# Autodesk Inventor assembly: ABD_RIGHT_OP
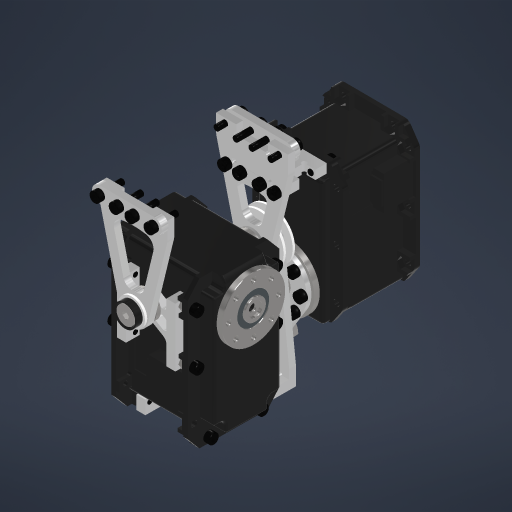
[picture p0: Inventor's stored thumbnail of the model, 512x512]
Saved by Autodesk Inventor 2024.3 (Build 283343000, 343)
## iProperties
Created: 2024-01-25
Part Number: ABD_RIGHT_OP
Document SubType Name: Assembly
Designer: ASUS
Mass: 367.451 g
Surface Area: 648.88 cm^2
Volume: 184.634 cm^3
Author: ASUS
## Documents named in this file (21)
- C:\Users\ASUS\Desktop\Anti_Backlash_Structure_OP\v1_Frame\ABD_RIGHT_OP.iam
- C:\Users\ASUS\Desktop\Anti_Backlash_Structure_OP\v1_Frame\Roll_Fixation_R.ipt
- C:\Users\ASUS\Desktop\Anti_Backlash_Structure_OP\v1_Frame\Slider_crank_horn.ipt
- C:\Users\ASUS\Desktop\Anti_Backlash_Structure_OP\v1_Frame\Roll_Fixation_L.ipt
- C:\Users\ASUS\Desktop\Anti_Backlash_Structure_OP\v1_Frame\Roll_Fixation_Frame.ipt
- C:\Users\ASUS\Desktop\Anti_Backlash_Structure_OP\v1_Frame\Leg_joint_slider_frame.ipt
- C:\Users\ASUS\Desktop\Anti_Backlash_Structure_OP\v1_Frame\Roll_Fixation_Frame_Back.ipt
- C:\Users\ASUS\Desktop\Anti_Backlash_Structure_OP\v1_Frame\106_Slider_Fixation.ipt
- C:\Users\ASUS\Desktop\Anti_Backlash_Structure_OP\v1_Frame\hip joint fix washer.ipt
- C:\Users\ASUS\Desktop\Anti_Backlash_Structure_OP\v1_Frame\Roll_Fixation_Frameto64.ipt
- C:\Users\ASUS\Desktop\ABD_2024_Eindhoven\MISUMI\Roll_Fixation_Frame_8mm_Set.iam
- C:\Users\ASUS\Desktop\ABD_2024_Eindhoven\MISUMI\CSH-ST-M2_5-8_203.ipt
- C:\Users\ASUS\Desktop\ABD_2024_Eindhoven\MISUMI\hip_joint_fix_washer_10mm_Set.iam
- C:\Users\ASUS\Desktop\Anti_Backlash_Structure_OP\MISUMI\ABD_4mm_set.iam
- C:\Users\ASUS\Desktop\Anti_Backlash_Structure_OP\v1_Frame\Front_Frame_Fixer.iam
- C:\Users\ASUS\Desktop\Anti_Backlash_Structure_OP\v1_Frame\Rear_Frame_Fixer.iam
- C:\Users\ASUS\Desktop\Anti_Backlash_Structure_OP\v1_Frame\Crank_Slider_Fixer.iam
- C:\Users\ASUS\Desktop\Anti_Backlash_Structure_OP\ROBOTIS(Inventor 2024 ver.)\DXL\MX-106T+idle.ipt.iam
- C:\Users\ASUS\Desktop\Anti_Backlash_Structure_OP\ROBOTIS(Inventor 2024 ver.)\DXL\MX-64T.ipt
- C:\Users\ASUS\Desktop\ABD_2024_Eindhoven\ROBOTIS(Inventor 2024 ver.)\HORN\64-106Horn.ipt
- MX-106T+idle.ipt
## Components (30 placed, 19 different names)
1. Roll_Fixation_R:1 — 메이트:51, 각도:1, 삽입:2, 삽입:24, 메이트:76
2. Slider_crank_horn:1 — 삽입:3, 삽입:20, 메이트:69, 삽입:29, 메이트:82
3. Roll_Fixation_L:1 — 메이트:52, 각도:2, 삽입:4, 메이트:77
4. Roll_Fixation_Frame:1 — 메이트:51, 메이트:54
5. Leg_joint_slider_frame:1 — 메이트:53, 삽입:17, 삽입:18, 메이트:63, 메이트:83
6. Roll_Fixation_Frame_Back:1 — 메이트:52, 메이트:53, 플러쉬:1, 삽입:13, 삽입:16, 각도:3, 삽입:23
7. 106_Slider_Fixation:1 — 메이트:72, 메이트:73, 메이트:74
8. hip joint fix washer:1 — 삽입:5, 메이트:55
9. hip joint fix washer:2 — 삽입:6, 메이트:56
10. Roll_Fixation_Frameto64:1 — 플러쉬:1, 삽입:14, 삽입:15, 메이트:66, 메이트:68, 메이트:80, 메이트:81
11. Roll_Fixation_Frame_8mm_Set:1 [sub-assembly] — 메이트:77, 메이트:78, 삽입:25
12. Roll_Fixation_Frame_8mm_Set:2 [sub-assembly] — 삽입:22, 메이트:75
13. CSH-ST-M2_5-8_203:1 — 삽입:18
14. CSH-ST-M2_5-8_203:2 — 삽입:17
15. Roll_Fixation_Frame_8mm_Set:3 [sub-assembly] — 삽입:26, 메이트:79
16. hip_joint_fix_washer_10mm_Set:1 [sub-assembly] — 삽입:5, 메이트:55
17. hip_joint_fix_washer_10mm_Set:2 [sub-assembly] — 삽입:6, 메이트:56
18. CSH-ST-M2_5-8_203:3 — 삽입:15
19. CSH-ST-M2_5-8_203:4 — 삽입:13
20. CSH-ST-M2_5-8_203:5 — 삽입:14
21. CSH-ST-M2_5-8_203:6 — 삽입:16
22. Front_Frame_Fixer:1 [sub-assembly] — 각도:1, 삽입:2, 메이트:54
23. Rear_Frame_Fixer:1 [sub-assembly] — 각도:2, 삽입:4, 삽입:23
24. Crank_Slider_Fixer:1 [sub-assembly] — 삽입:3, 메이트:63, 메이트:83
25. CSH-ST-M2_5-8_203:7 — 메이트:66, 삽입:27
26. CSH-ST-M2_5-8_203:8 — 메이트:68, 삽입:28
27. ABD_4mm_set:1 [sub-assembly] — 삽입:20, 메이트:69
28. MX-106T+idle.ipt:1 [sub-assembly] — 메이트:72, 메이트:73, 메이트:74, 삽입:22, 메이트:75, 삽입:24, 메이트:76, 메이트:78, 삽입:25, 삽입:26, 메이트:79
29. MX-64T:1 — 메이트:80, 메이트:81, 삽입:27, 삽입:28
30. 64-106Horn:1 — 삽입:29, 메이트:82
## Relationships (59: Mate 34, Insert 21, Angle 3, Flush 1)
- [Mate]: Roll_Fixation_Frame:1 ↔ Roll_Fixation_Frame_Back:1
- [Mate]: Leg_joint_slider_frame:1 ↔ 106_Slider_Fixation:1
- [Mate]: Leg_joint_slider_frame:1 ↔ 106_Slider_Fixation:1
- [Mate]: Leg_joint_slider_frame:1 ↔ 106_Slider_Fixation:1
- [Mate]: Roll_Fixation_Frame:1 ↔ hip joint fix washer:1
- [Mate]: Roll_Fixation_Frame:1 ↔ hip joint fix washer:1
- [Mate]: Roll_Fixation_Frame:1 ↔ hip joint fix washer:1
- [Mate]: Roll_Fixation_Frame_Back:1 ↔ hip joint fix washer:2
- [Mate]: Roll_Fixation_Frame_Back:1 ↔ hip joint fix washer:2
- [Mate]: Roll_Fixation_Frame_Back:1 ↔ hip joint fix washer:2
- [Mate]: Roll_Fixation_Frame_Back:1 ↔ Roll_Fixation_Frameto64:1
- [Mate]: Roll_Fixation_Frame_Back:1 ↔ Roll_Fixation_Frameto64:1
- 메이트:51 [Mate]: Roll_Fixation_R:1 ↔ Roll_Fixation_Frame:1
- 메이트:52 [Mate]: Roll_Fixation_L:1 ↔ Roll_Fixation_Frame_Back:1
- 메이트:53 [Mate]: Leg_joint_slider_frame:1 ↔ Roll_Fixation_Frame_Back:1
- 각도:1 [Angle] (0 deg): Roll_Fixation_R:1 ↔ Front_Frame_Fixer:1
- 삽입:2 [Insert]: Roll_Fixation_R:1 ↔ Front_Frame_Fixer:1
- 삽입:3 [Insert]: Slider_crank_horn:1 ↔ Crank_Slider_Fixer:1
- 각도:2 [Angle] (0 deg): Roll_Fixation_L:1 ↔ Rear_Frame_Fixer:1
- 삽입:4 [Insert]: Roll_Fixation_L:1 ↔ Rear_Frame_Fixer:1
- 메이트:54 [Mate]: Roll_Fixation_Frame:1 ↔ Front_Frame_Fixer:1
- 삽입:5 [Insert]: hip joint fix washer:1 ↔ hip_joint_fix_washer_10mm_Set:1
- 메이트:55 [Mate]: hip joint fix washer:1 ↔ hip_joint_fix_washer_10mm_Set:1
- 삽입:6 [Insert]: hip joint fix washer:2 ↔ hip_joint_fix_washer_10mm_Set:2
- 메이트:56 [Mate]: hip joint fix washer:2 ↔ hip_joint_fix_washer_10mm_Set:2
- 플러쉬:1 [Flush]: Roll_Fixation_Frame_Back:1 ↔ Roll_Fixation_Frameto64:1
- 삽입:13 [Insert]: Roll_Fixation_Frame_Back:1 ↔ CSH-ST-M2_5-8_203:4
- 삽입:14 [Insert]: Roll_Fixation_Frameto64:1 ↔ CSH-ST-M2_5-8_203:5
- 삽입:15 [Insert]: Roll_Fixation_Frameto64:1 ↔ CSH-ST-M2_5-8_203:3
- 삽입:16 [Insert]: Roll_Fixation_Frame_Back:1 ↔ CSH-ST-M2_5-8_203:6
- 삽입:17 [Insert]: Leg_joint_slider_frame:1 ↔ CSH-ST-M2_5-8_203:2
- 삽입:18 [Insert]: Leg_joint_slider_frame:1 ↔ CSH-ST-M2_5-8_203:1
- 메이트:63 [Mate]: Leg_joint_slider_frame:1 ↔ Crank_Slider_Fixer:1
- 메이트:66 [Mate]: Roll_Fixation_Frameto64:1 ↔ CSH-ST-M2_5-8_203:7
- 메이트:68 [Mate]: Roll_Fixation_Frameto64:1 ↔ CSH-ST-M2_5-8_203:8
- 삽입:20 [Insert]: Slider_crank_horn:1 ↔ ABD_4mm_set:1
- 메이트:69 [Mate]: Slider_crank_horn:1 ↔ ABD_4mm_set:1
- 각도:3 [Angle] (0 deg): Roll_Fixation_Frame_Back:1
- [Insert] (0.5 mm): MX-64T:1 ↔ 64-106Horn:1
- 메이트:72 [Mate]: 106_Slider_Fixation:1 ↔ MX-106T+idle.ipt:1
- 메이트:73 [Mate]: 106_Slider_Fixation:1 ↔ MX-106T+idle.ipt:1
- 메이트:74 [Mate] (0.5 mm): 106_Slider_Fixation:1 ↔ MX-106T+idle.ipt:1
- 삽입:22 [Insert]: Roll_Fixation_Frame_8mm_Set:2 ↔ MX-106T+idle.ipt:1
- 메이트:75 [Mate]: Roll_Fixation_Frame_8mm_Set:2 ↔ MX-106T+idle.ipt:1
- 삽입:23 [Insert]: Roll_Fixation_Frame_Back:1 ↔ Rear_Frame_Fixer:1
- 삽입:24 [Insert] (0.5 mm): Roll_Fixation_R:1 ↔ MX-106T+idle.ipt:1
- 메이트:76 [Mate]: Roll_Fixation_R:1 ↔ MX-106T+idle.ipt:1
- 메이트:77 [Mate]: Roll_Fixation_L:1 ↔ Roll_Fixation_Frame_8mm_Set:1
- 메이트:78 [Mate]: Roll_Fixation_Frame_8mm_Set:1 ↔ MX-106T+idle.ipt:1
- 삽입:25 [Insert]: Roll_Fixation_Frame_8mm_Set:1 ↔ MX-106T+idle.ipt:1
- 삽입:26 [Insert]: Roll_Fixation_Frame_8mm_Set:3 ↔ MX-106T+idle.ipt:1
- 메이트:79 [Mate]: Roll_Fixation_Frame_8mm_Set:3 ↔ MX-106T+idle.ipt:1
- 메이트:80 [Mate]: Roll_Fixation_Frameto64:1 ↔ MX-64T:1
- 메이트:81 [Mate]: Roll_Fixation_Frameto64:1 ↔ MX-64T:1
- 삽입:27 [Insert]: CSH-ST-M2_5-8_203:7 ↔ MX-64T:1
- 삽입:28 [Insert]: CSH-ST-M2_5-8_203:8 ↔ MX-64T:1
- 삽입:29 [Insert]: Slider_crank_horn:1 ↔ 64-106Horn:1
- 메이트:82 [Mate]: Slider_crank_horn:1 ↔ 64-106Horn:1
- 메이트:83 [Mate]: Leg_joint_slider_frame:1 ↔ Crank_Slider_Fixer:1
